# Autodesk Inventor assembly: OmniPod
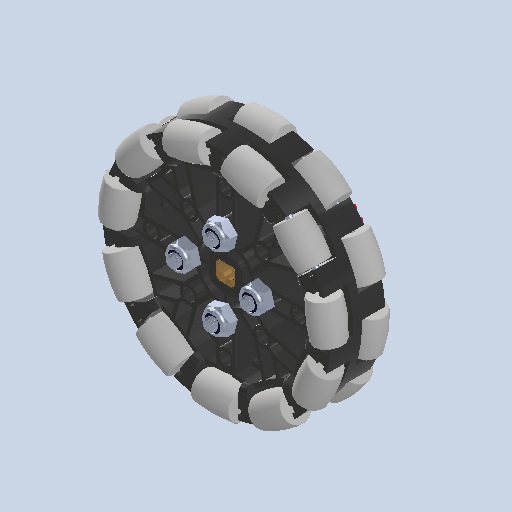
[picture p0: Inventor's stored thumbnail of the model, 512x512]
Saved by Autodesk Inventor 2025.1 (Build 291241020, 241B)
## iProperties
Created: 2024-10-26
Part Number: OmniPod
Document SubType Name: Assembly
Designer: Juan
Author: Juan
## Documents named in this file (9)
- C:\Users\Hunter Mathis\Documents\GitHub\ATUM-V5RC-High-Stakes-CAD\Robot\Subassemblies\OmniPod.iam
- C:\Users\Hunter Mathis\Documents\GitHub\ATUM-V5RC-High-Stakes-CAD\VEX-CAD-Inventor\Motion\Wheels\Omni Wheel\3.25 Omni AS, No Insert.iam
- C:\Users\Juan\Documents\GitHub\ATUM-VRC-High-Stakes-CAD\VEX-CAD-Inventor\Motion\Wheels\Omni Wheel.iam
- C:\Users\Hunter Mathis\Documents\GitHub\ATUM-V5RC-High-Stakes-CAD\VEX-CAD-Inventor\Motion\Gears\HS Gear\HS 48T Gear, Circle.iam
- C:\Users\Juan\Documents\GitHub\ATUM-VRC-High-Stakes-CAD\VEX-CAD-Inventor\Motion\Gears\HS Gear.iam
- C:\Users\Hunter Mathis\Documents\GitHub\ATUM-V5RC-High-Stakes-CAD\VEX-CAD-Inventor\Structure\Hardware\Screw Steel - Star\SScrew Star Threaded 1.250.ipt
- C:\Users\Juan\Documents\GitHub\ATUM-VRC-High-Stakes-CAD\VEX-CAD-Inventor\Structure\Hardware\Screw Steel - Star.ipt
- C:\Users\Hunter Mathis\Documents\GitHub\ATUM-V5RC-High-Stakes-CAD\VEX-CAD-Inventor\Structure\Hardware\Nut Thin Nylock.ipt
- C:\Users\Hunter Mathis\Documents\GitHub\ATUM-V5RC-High-Stakes-CAD\VEX-CAD-Inventor\Motion\HS Shaft Adapter Circle.ipt
## Components (11 placed, 5 different names)
1. 3.25 Omni AS, No Insert:1 [sub-assembly] — Mate:1, Mate:2, Mate:3, Mate:4, Mate:5, Mate:9, Mate:10, Mate:11, Mate:12, Flush:1
2. HS 48T Gear, Circle:1 [sub-assembly] — Mate:1, Mate:2, Mate:3, Mate:4, Mate:5, Mate:6, Mate:7
3. HS Shaft Adapter Circle:1 — Mate:10, Mate:11, Mate:12, Flush:1
4. SScrew Star Threaded 1.250:1 — Mate:6, Mate:7, Mate:8
5. Nut Thin Nylock:1 — Mate:8, Mate:9
6. SScrew Star Threaded 1.250:2
7. Nut Thin Nylock:2
8. SScrew Star Threaded 1.250:3
9. Nut Thin Nylock:3
10. SScrew Star Threaded 1.250:4
11. Nut Thin Nylock:4
## Component patterns: (4 elements, first: SScrew Star Threaded 1.250:1 + Nut Thin Nylock:1)
## Relationships (13: Mate 12, Flush 1)
- Mate:1: 3.25 Omni AS, No Insert:1 ↔ HS 48T Gear, Circle:1
- Mate:2: 3.25 Omni AS, No Insert:1 ↔ HS 48T Gear, Circle:1
- Mate:3: 3.25 Omni AS, No Insert:1 ↔ HS 48T Gear, Circle:1
- Mate:4: 3.25 Omni AS, No Insert:1 ↔ HS 48T Gear, Circle:1
- Mate:5: 3.25 Omni AS, No Insert:1 ↔ HS 48T Gear, Circle:1
- Mate:6: HS 48T Gear, Circle:1 ↔ SScrew Star Threaded 1.250:1
- Mate:7: HS 48T Gear, Circle:1 ↔ SScrew Star Threaded 1.250:1
- Mate:8: SScrew Star Threaded 1.250:1 ↔ Nut Thin Nylock:1
- Mate:9: 3.25 Omni AS, No Insert:1 ↔ Nut Thin Nylock:1
- Mate:10: 3.25 Omni AS, No Insert:1 ↔ HS Shaft Adapter Circle:1
- Mate:11: 3.25 Omni AS, No Insert:1 ↔ HS Shaft Adapter Circle:1
- Mate:12: 3.25 Omni AS, No Insert:1 ↔ HS Shaft Adapter Circle:1
- Flush:1: 3.25 Omni AS, No Insert:1 ↔ HS Shaft Adapter Circle:1
